# Autodesk Inventor assembly: Ensamblaje carro
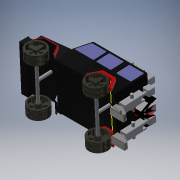
[picture p0: Inventor's stored thumbnail of the model, 180x180]
Saved by Autodesk Inventor 2017 (Build 210142000, 142)
## iProperties
Part Number: Ensamblaje carro
Material: Genérico
Document SubType Name: Assembly
Designer: HOME
Author: HOME
## Documents named in this file (9)
- C:\Users\HOME\Desktop\Transformer\Transformer\Ensamblaje carro.iam
- C:\Users\HOME\Desktop\Transformer\Transformer\Carro\Bumper.ipt
- C:\Users\HOME\Desktop\Transformer\Transformer\NuevoProyecto\PuertaMarco.iam
- C:\Users\HOME\Downloads\llanta xddd.ipt
- C:\Users\HOME\Desktop\Transformer\Transformer\Hombro.ipt
- C:\Users\HOME\Desktop\Transformer\Transformer\Union pie.ipt
- C:\Users\HOME\Desktop\Transformer\Transformer\Ante pierna.ipt
- C:\Users\HOME\Desktop\Transformer\Transformer\Pie.ipt
- C:\Users\HOME\Desktop\Transformer\Transformer\CabezaCarro.ipt
## Components (23 placed, 8 different names)
1. PuertaMarco:1 [sub-assembly] — Rígido:17, De rotación:6, De rotación:8, Rígido:1, Rígido:2, Rígido:6, Rígido:7, Rígido:16
2. Bumper:1 — Rígido:17, De rotación:5, De rotación:7
3. llanta xddd:2 — De rotación:5
4. llanta xddd:3 — De rotación:6
5. llanta xddd:4 — De rotación:7
6. llanta xddd:5 — De rotación:8
7. Hombro:2 — Rígido:1, Insertar:1
8. Hombro:3 — Rígido:2, Rígido:3
9. Union pie:1 — Rígido:3, Rígido:4
10. Union pie:2 — Insertar:1, Rígido:5
11. Ante pierna:1 — Rígido:4
12. Ante pierna:2 — Rígido:5
13. Hombro:4 — Rígido:6, Rígido:9
14. Hombro:5 — Rígido:7, Rígido:8
15. Union pie:3 — Rígido:8, Rígido:10
16. Union pie:4 — Rígido:9, Rígido:11
17. Ante pierna:3 — Rígido:11, Rígido:12
18. Ante pierna:4 — Rígido:10, Rígido:13
19. Union pie:5 — Rígido:13, Rígido:15
20. Union pie:6 — Rígido:12, Rígido:14
21. Pie:1 — Rígido:15
22. Pie:2 — Rígido:14
23. CabezaCarro:1 — Rígido:16
## Relationships (22: WeldJoint 17, RevoluteJoint 4, Insert 1)
- Rígido:17 [WeldJoint]: PuertaMarco:1 ↔ Bumper:1
- De rotación:5 [RevoluteJoint]: Bumper:1 ↔ llanta xddd:2
- De rotación:6 [RevoluteJoint]: PuertaMarco:1 ↔ llanta xddd:3
- De rotación:7 [RevoluteJoint]: Bumper:1 ↔ llanta xddd:4
- De rotación:8 [RevoluteJoint]: PuertaMarco:1 ↔ llanta xddd:5
- Rígido:1 [WeldJoint]: PuertaMarco:1 ↔ Hombro:2
- Rígido:2 [WeldJoint]: PuertaMarco:1 ↔ Hombro:3
- Rígido:3 [WeldJoint]: Hombro:3 ↔ Union pie:1
- Insertar:1: Hombro:2 ↔ Union pie:2
- Rígido:4 [WeldJoint]: Union pie:1 ↔ Ante pierna:1
- Rígido:5 [WeldJoint]: Union pie:2 ↔ Ante pierna:2
- Rígido:6 [WeldJoint]: PuertaMarco:1 ↔ Hombro:4
- Rígido:7 [WeldJoint]: PuertaMarco:1 ↔ Hombro:5
- Rígido:8 [WeldJoint]: Hombro:5 ↔ Union pie:3
- Rígido:9 [WeldJoint]: Hombro:4 ↔ Union pie:4
- Rígido:10 [WeldJoint]: Union pie:3 ↔ Ante pierna:4
- Rígido:11 [WeldJoint]: Union pie:4 ↔ Ante pierna:3
- Rígido:12 [WeldJoint]: Ante pierna:3 ↔ Union pie:6
- Rígido:13 [WeldJoint]: Ante pierna:4 ↔ Union pie:5
- Rígido:14 [WeldJoint]: Union pie:6 ↔ Pie:2
- Rígido:15 [WeldJoint]: Union pie:5 ↔ Pie:1
- Rígido:16 [WeldJoint]: PuertaMarco:1 ↔ CabezaCarro:1
